# Autodesk Inventor assembly: Assembly1
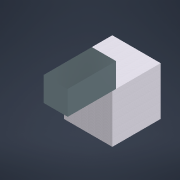
[picture p0: Inventor's stored thumbnail of the model, 180x180]
Saved by Autodesk Inventor 2021 (Build 250183000, 183)
## iProperties
Created: 2021-12-26
Part Number: Assembly1
Document SubType Name: Assembly
Designer: This-PC
Author: This-PC
## Documents named in this file (3)
- G:\Projects\Project 001\Inventor\Assembly1.iam
- G:\Projects\Project 001\Inventor\Part1.ipt
- G:\Projects\Project 001\Inventor\Part2.ipt
## Components (2 placed, 2 different names)
1. Part1:1 — Mate:1
2. Part2:1 — Mate:1
## Relationships (1: Mate 1)
- Mate:1: Part1:1 ↔ Part2:1
